# Autodesk Inventor assembly: 99385c01
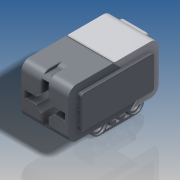
[picture p0: Inventor's stored thumbnail of the model, 180x180]
Saved by Autodesk Inventor 2016 SP2 (Build 200236200, 236)
## iProperties
Created: 2015-08-28
Part Number: 99385c01
Document SubType Name: Assembly
Designer: D. Kohfeld
Mass: 10.5068 g
Surface Area: 161.941 cm^2
Volume: 9.9121 cm^3
Density: 1.06 g/cm^3
Author: D. Kohfeld
## Documents named in this file (5)
- A:\LEGO Pieces\EV3\99385c01.iam
- A:\LEGO Pieces\EV3\99377-LtBluishGray.ipt
- A:\LEGO Pieces\EV3\99376-White.ipt
- A:\LEGO Pieces\EV3\54732b-LtBluishGray.ipt
- A:\LEGO Pieces\EV3\99385-LtBluishGray.ipt
## Components (4 placed, 4 different names)
1. 99377-LtBluishGray:1 — Flush:1, Flush:2, Mate:1, Mate:2, Mate:3, Mate:4
2. 99376-White:1 — Flush:1, Flush:3, Mate:3, Mate:5, Flush:4
3. 54732b-LtBluishGray:1 — Mate:4, Mate:5, Flush:4
4. 99385-LtBluishGray:1 — Flush:2, Mate:1, Mate:2, Flush:3
## Relationships (9: Mate 5, Flush 4)
- Flush:1: 99377-LtBluishGray:1 ↔ 99376-White:1
- Flush:2: 99377-LtBluishGray:1 ↔ 99385-LtBluishGray:1
- Mate:1: 99377-LtBluishGray:1 ↔ 99385-LtBluishGray:1
- Mate:2: 99377-LtBluishGray:1 ↔ 99385-LtBluishGray:1
- Flush:3: 99376-White:1 ↔ 99385-LtBluishGray:1
- Mate:3: 99377-LtBluishGray:1 ↔ 99376-White:1
- Mate:4: 99377-LtBluishGray:1 ↔ 54732b-LtBluishGray:1
- Mate:5: 99376-White:1 ↔ 54732b-LtBluishGray:1
- Flush:4: 99376-White:1 ↔ 54732b-LtBluishGray:1
